# Autodesk Inventor assembly: Chessboard Bottom
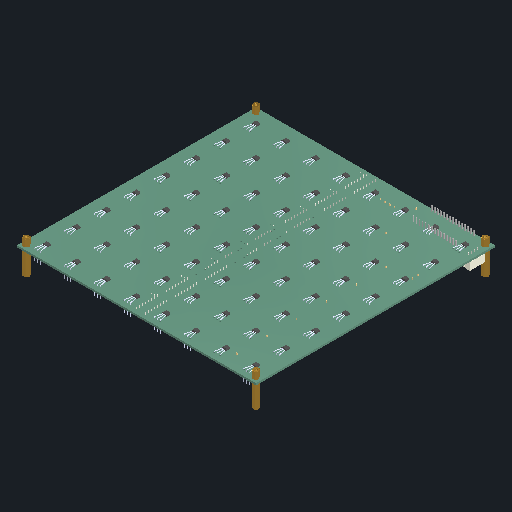
[picture p0: Inventor's stored thumbnail of the model, 512x512]
Saved by Autodesk Inventor 2026 (Build 300175000, 175)
## iProperties
Created: 2025-04-19
Part Number: Chessboard Bottom
Document SubType Name: Assembly
Designer: ckyiu
Author: ckyiu
## Documents named in this file (4)
- C:\Users\ckyiu\Documents\Projects\Chessboard-Design\Assemblies\Chessboard Bottom.iam
- C:\Users\ckyiu\Documents\Projects\Chessboard-Design\Assemblies\PCBs\Chessboard Hardware Model.iam
- C:\Users\ckyiu\Documents\Projects\Chessboard-Design\Parts\Standoffs\M2.5 F-F Standoff 6mm.ipt
- C:\Users\ckyiu\Documents\Projects\Chessboard-Design\Parts\Standoffs\M2.5 F-M Standoff 20mm.ipt
## Components (9 placed, 3 different names)
1. Chessboard Hardware Model:1 [sub-assembly] — Insert:1, Insert:2, Insert:3, Insert:4, Angle:1, Angle:2, Angle:3, Angle:4, Insert:5, Insert:6, Insert:7, Insert:8, Angle:5, Angle:6, Angle:7, Angle:8
2. M2.5 F-F Standoff 6mm:1 — Insert:1, Angle:1
3. M2.5 F-F Standoff 6mm:2 — Insert:2, Angle:2
4. M2.5 F-F Standoff 6mm:3 — Insert:3, Angle:3
5. M2.5 F-F Standoff 6mm:4 — Insert:4, Angle:4
6. M2.5 F-M Standoff 20mm:1 — Insert:5, Angle:5
7. M2.5 F-M Standoff 20mm:2 — Insert:6, Angle:6
8. M2.5 F-M Standoff 20mm:3 — Insert:7, Angle:7
9. M2.5 F-M Standoff 20mm:4 — Insert:8, Angle:8
## Relationships (16: Insert 8, Angle 8)
- Insert:1: Chessboard Hardware Model:1 ↔ M2.5 F-F Standoff 6mm:1
- Insert:2: Chessboard Hardware Model:1 ↔ M2.5 F-F Standoff 6mm:2
- Insert:3: Chessboard Hardware Model:1 ↔ M2.5 F-F Standoff 6mm:3
- Insert:4: Chessboard Hardware Model:1 ↔ M2.5 F-F Standoff 6mm:4
- Angle:1 (0 deg): Chessboard Hardware Model:1 ↔ M2.5 F-F Standoff 6mm:1
- Angle:2 (0 deg): Chessboard Hardware Model:1 ↔ M2.5 F-F Standoff 6mm:2
- Angle:3 (0 deg): Chessboard Hardware Model:1 ↔ M2.5 F-F Standoff 6mm:3
- Angle:4 (0 deg): Chessboard Hardware Model:1 ↔ M2.5 F-F Standoff 6mm:4
- Insert:5: Chessboard Hardware Model:1 ↔ M2.5 F-M Standoff 20mm:1
- Insert:6: Chessboard Hardware Model:1 ↔ M2.5 F-M Standoff 20mm:2
- Insert:7: Chessboard Hardware Model:1 ↔ M2.5 F-M Standoff 20mm:3
- Insert:8: Chessboard Hardware Model:1 ↔ M2.5 F-M Standoff 20mm:4
- Angle:5 (0 deg): Chessboard Hardware Model:1 ↔ M2.5 F-M Standoff 20mm:1
- Angle:6 (0 deg): Chessboard Hardware Model:1 ↔ M2.5 F-M Standoff 20mm:2
- Angle:7 (0 deg): Chessboard Hardware Model:1 ↔ M2.5 F-M Standoff 20mm:3
- Angle:8 (0 deg): Chessboard Hardware Model:1 ↔ M2.5 F-M Standoff 20mm:4
